# Autodesk Inventor assembly: fab_model_mk-2[1]
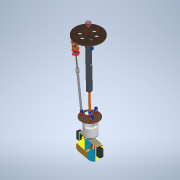
[picture p0: Inventor's stored thumbnail of the model, 180x180]
Saved by Autodesk Inventor 2021 (Build 250183000, 183)
## iProperties
Created: 2020-12-19
Part Number: fab_model_mk-2[1]
Document SubType Name: Assembly
Designer: Vikki
Author: Vikki
## Documents named in this file (31)
- E:\UG projects\CTF- projects\BOREWELL RESCUER\borewell rescuebot 2021\pll manipulator files\sps manipulator\fab_model_mk-2 scavenger bot.iam
- E:\UG projects\CTF- projects\BOREWELL RESCUER\borewell rescuebot 2021\pll manipulator files\sps manipulator\base.ipt
- E:\UG projects\CTF- projects\BOREWELL RESCUER\borewell rescuebot 2021\pll manipulator files\sps manipulator\craftsman-3-pc-universal-joint-set-1.snapshot.1\Craftsman Socket U-Joint.iam
- E:\UG projects\CTF- projects\BOREWELL RESCUER\borewell rescuebot 2021\pll manipulator files\sps manipulator\platform.ipt
- E:\UG projects\CTF- projects\BOREWELL RESCUER\borewell rescuebot 2021\pll manipulator files\sps manipulator\leadscrew.ipt
- E:\UG projects\CTF- projects\BOREWELL RESCUER\borewell rescuebot 2021\pll manipulator files\sps manipulator\coupler.ipt
- E:\UG projects\CTF- projects\BOREWELL RESCUER\borewell rescuebot 2021\pll manipulator files\sps manipulator\telescopic boom1.ipt
- E:\UG projects\CTF- projects\BOREWELL RESCUER\borewell rescuebot 2021\pll manipulator files\sps manipulator\boom 3.ipt
- E:\UG projects\CTF- projects\BOREWELL RESCUER\borewell rescuebot 2021\pll manipulator files\sps manipulator\ball-pin.ipt
- E:\UG projects\CTF- projects\BOREWELL RESCUER\borewell rescuebot 2021\2020 bot\borewell max sixe.ipt
- E:\UG projects\CTF- projects\BOREWELL RESCUER\borewell rescuebot 2021\2020 bot\min size bore well.ipt
- E:\UG projects\CTF- projects\BOREWELL RESCUER\borewell rescuebot 2021\pll manipulator files\sps manipulator\MicroGearmotor v3.ipt
- E:\UG projects\CTF- projects\BOREWELL RESCUER\borewell rescuebot 2021\pll manipulator files\sps manipulator\plunger.ipt
- E:\UG projects\CTF- projects\BOREWELL RESCUER\borewell rescuebot 2021\pll manipulator files\sps manipulator\piston.ipt
- E:\UG projects\CTF- projects\BOREWELL RESCUER\borewell rescuebot 2021\pll manipulator files\sps manipulator\motor bracket n 20.ipt
- E:\UG projects\CTF- projects\BOREWELL RESCUER\borewell rescuebot 2021\pll manipulator files\sps manipulator\female joint for uv.ipt
- E:\UG projects\CTF- projects\BOREWELL RESCUER\borewell rescuebot 2021\pll manipulator files\sps manipulator\platform uv femal joint.ipt
- E:\UG projects\CTF- projects\BOREWELL RESCUER\borewell rescuebot 2021\pll manipulator files\sps manipulator\boom to female.ipt
- E:\UG projects\CTF- projects\BOREWELL RESCUER\borewell rescuebot 2021\pll manipulator files\sps manipulator\fab_model_mk-2[1]\Design Accelerator\Bearing1.iam
- E:\UG projects\CTF- projects\BOREWELL RESCUER\borewell rescuebot 2021\pll manipulator files\sps manipulator\z axis-motor coupling.ipt
- E:\UG projects\CTF- projects\BOREWELL RESCUER\borewell rescuebot 2021\pll manipulator files\sps manipulator\jack-pin.ipt
- E:\UG projects\CTF- projects\BOREWELL RESCUER\borewell rescuebot 2021\pll manipulator files\sps manipulator\kiso.ipt
- E:\UG projects\CTF- projects\BOREWELL RESCUER\borewell rescuebot 2021\pll manipulator files\sps manipulator\new-motor-base.ipt
- E:\UG projects\CTF- projects\BOREWELL RESCUER\borewell rescuebot 2021\pll manipulator files\sps manipulator\end eff servo-conector.ipt
- E:\UG projects\CTF- projects\BOREWELL RESCUER\borewell rescuebot 2021\pll manipulator files\sps manipulator\clamshell half.ipt
- E:\UG projects\CTF- projects\BOREWELL RESCUER\borewell rescuebot 2021\pll manipulator files\sps manipulator\clamshell half-2.ipt
- E:\UG projects\CTF- projects\BOREWELL RESCUER\borewell rescuebot 2021\pll manipulator files\sps manipulator\clamshell cross link.ipt
- E:\UG projects\CTF- projects\BOREWELL RESCUER\borewell rescuebot 2021\pll manipulator files\sps manipulator\clamsheel sheet surface.ipt
- E:\UG projects\CTF- projects\BOREWELL RESCUER\borewell rescuebot 2021\pll manipulator files\sps manipulator\fab_model_mk-2[1]\Design Accelerator\Bearing3.iam
- E:\UG projects\CTF- projects\BOREWELL RESCUER\borewell rescuebot 2021\pll manipulator files\sps manipulator\n20 motor 3dp support.ipt
- E:\UG projects\CTF- projects\BOREWELL RESCUER\borewell rescuebot 2021\pll manipulator files\sps manipulator\z axis motor cover.ipt
## Components (45 placed, 29 different names)
1. base:1 — Mate:1, Mate:2, Mate:3, Mate:4, Mate:5, Mate:6, Angle:1, Mate:18, Mate:19, Mate:61, Flush:6, M1 C, M2 C, Mate:150, Mate:151
2. Craftsman Socket U-Joint:1 [sub-assembly] — Mate:1, Mate:2, Angle:2, Mate:90
3. Craftsman Socket U-Joint:2 [sub-assembly] — Mate:5, Mate:6, Angle:3, Mate:92
4. Craftsman Socket U-Joint:3 [sub-assembly] — Mate:3, Mate:4, Angle:1, Angle:2, Angle:3, Mate:23, Mate:91, Mate:93, Angle:7, Mate:108, Mate:109
5. platform:1 — Mate:7, Mate:9, Mate:10, Mate:16, Mate:17, M1 C, M2 C, Angle:6, Mate:134, Mate:135, Mate:136, Mate:199, Mate:200, Mate:201, Mate:204, Mate:205
6. Craftsman Socket U-Joint:4 [sub-assembly] — Mate:7, Mate:90, Mate:135
7. Craftsman Socket U-Joint:5 [sub-assembly] — Mate:9, Mate:91, Mate:111, Mate:112, Mate:136
8. Craftsman Socket U-Joint:6 [sub-assembly] — Mate:10, Mate:23, Mate:92, Mate:134
9. Craftsman Socket U-Joint:7 [sub-assembly] — Mate:16, Mate:17, Mate:26, Flush:1, Mate:60, Angle:6, Mate:100, Mate:101
10. Craftsman Socket U-Joint:8 [sub-assembly] — Mate:18, Mate:19, Angle:5, Mate:26, Flush:1, Mate:48, Mate:59, Mate:114, Mate:115
11. leadscrew:1 — Mate:97, Mate:167, Mate:187, Mate:188
12. telescopic boom1:1 — Mate:48, Mate:59, Angle:12
13. boom 3:1 — Mate:100, Mate:101, Angle:12
14. ball-pin:1 — Mate:60
15. borewell max sixe:1 — Mate:61, Mate:62, Flush:5
16. min size bore well:1 — Mate:62, Flush:5, Flush:6
17. MicroGearmotor v3:1 — Mate:93, Angle:7, Angle:9, Mate:120, Mate:167
18. plunger:1 — Mate:97, Angle:11, Mate:113, Mate:137
19. piston:1 — Angle:10, Angle:11, Mate:117
20. motor bracket n 20:1 — Angle:9, Mate:110, Angle:10, Mate:117, Mate:120, Flush:26, Mate:203
21. female joint for uv:1 — Mate:108, Mate:109, Mate:110
22. platform uv femal joint:1 — Mate:111, Mate:112, Mate:113, Mate:137
23. boom to female:1 — Mate:114, Mate:115
24. coupler:2 — Mate:188, Mate:189
25. Bearing:6 [sub-assembly] — Mate:187, Flush:26, Mate:189
26. z axis-motor coupling:1 — Mate:152, Mate:153, Mate:190, Mate:204, Mate:205
27. jack-pin:1 — Mate:150, Mate:151, Mate:191, Flush:27
28. kiso:1 — Mate:157, Mate:162, Mate:163, Mate:168, Mate:169, Mate:170
29. new-motor-base:1 — Mate:152, Mate:153, Mate:157, Mate:168, Mate:169, Mate:171, Mate:172, Mate:190, Angle:14
30. kiso:2 — Mate:160, Mate:161, Mate:170, Mate:171, Mate:172
31. end eff servo-conector:1 — Mate:160, Mate:161, Mate:173, Mate:174
32. end eff servo-conector:2 — Mate:162, Mate:163, Mate:165, Mate:166
33. clamshell half:1 — Flush:14, Mate:164, Mate:165, Mate:166, Flush:17, Mate:177, Mate:179, Mate:186, Flush:20, Flush:21
34. clamshell half-2:1 — Flush:14, Mate:164, Flush:16, Mate:180, Mate:181, Mate:182, Mate:183, Flush:18
35. clamshell half:2 — Mate:173, Mate:174, Mate:175, Flush:15, Flush:16, Flush:22, Flush:23, Flush:24, Flush:25, Angle:14, Mate:192
36. clamshell half-2:2 — Mate:175, Flush:15, Flush:17, Mate:184, Mate:185, Mate:192
37. clamshell cross link:1 — Mate:177, Mate:184
38. clamshell cross link:2 — Mate:179, Mate:185
39. clamshell cross link:3 — Mate:180, Mate:181
40. clamshell cross link:4 — Mate:182, Mate:183
41. clamsheel sheet surface:1 — Flush:18, Flush:22, Flush:23, Flush:24, Flush:25
42. clamsheel sheet surface:2 — Mate:186, Flush:20, Flush:21
43. Bearing:7 [sub-assembly] — Mate:191, Flush:27
44. n20 motor 3dp support:1 — Mate:203
45. z axis motor cover:1 — Mate:199, Mate:200, Mate:201
## Relationships (114: Mate 84, Flush 19, Angle 11)
- Mate:1: base:1 ↔ Craftsman Socket U-Joint:1
- Mate:2: base:1 ↔ Craftsman Socket U-Joint:1
- Mate:3: base:1 ↔ Craftsman Socket U-Joint:3
- Mate:4: base:1 ↔ Craftsman Socket U-Joint:3
- Mate:5: base:1 ↔ Craftsman Socket U-Joint:2
- Mate:6: base:1 ↔ Craftsman Socket U-Joint:2
- Mate:7: platform:1 ↔ Craftsman Socket U-Joint:4
- Mate:9: platform:1 ↔ Craftsman Socket U-Joint:5
- Mate:10: platform:1 ↔ Craftsman Socket U-Joint:6
- Angle:1 (30 deg): base:1 ↔ Craftsman Socket U-Joint:3
- Angle:2 (60 deg): Craftsman Socket U-Joint:1 ↔ Craftsman Socket U-Joint:3
- Angle:3 (120 deg): Craftsman Socket U-Joint:2 ↔ Craftsman Socket U-Joint:3
- Mate:16: platform:1 ↔ Craftsman Socket U-Joint:7
- Mate:17: platform:1 ↔ Craftsman Socket U-Joint:7
- Mate:18: base:1 ↔ Craftsman Socket U-Joint:8
- Mate:19: base:1 ↔ Craftsman Socket U-Joint:8
- Angle:5 (0 deg): Craftsman Socket U-Joint:8
- Mate:23: Craftsman Socket U-Joint:3 ↔ Craftsman Socket U-Joint:6
- Mate:26: Craftsman Socket U-Joint:7 ↔ Craftsman Socket U-Joint:8
- Flush:1: Craftsman Socket U-Joint:7 ↔ Craftsman Socket U-Joint:8
- Mate:48: Craftsman Socket U-Joint:8 ↔ telescopic boom1:1
- Mate:59 (-5 mm): Craftsman Socket U-Joint:8 ↔ telescopic boom1:1
- Mate:60: Craftsman Socket U-Joint:7 ↔ ball-pin:1
- [Flush]: borewell max sixe:1 ↔ min size bore well:1
- [Flush]: borewell max sixe:1 ↔ min size bore well:1
- Mate:61: base:1 ↔ borewell max sixe:1
- Mate:62: borewell max sixe:1 ↔ min size bore well:1
- Flush:5: borewell max sixe:1 ↔ min size bore well:1
- Flush:6 (-400 mm): base:1 ↔ min size bore well:1
- M1 C [Flush] (400 mm): base:1 ↔ platform:1
- M2 C [Mate]: base:1 ↔ platform:1
- Mate:90: Craftsman Socket U-Joint:1 ↔ Craftsman Socket U-Joint:4
- Mate:91: Craftsman Socket U-Joint:3 ↔ Craftsman Socket U-Joint:5
- Mate:92: Craftsman Socket U-Joint:2 ↔ Craftsman Socket U-Joint:6
- Angle:6 (30 deg): platform:1 ↔ Craftsman Socket U-Joint:7
- Mate:93: Craftsman Socket U-Joint:3 ↔ MicroGearmotor v3:1
- Angle:7 (0 deg): Craftsman Socket U-Joint:3 ↔ MicroGearmotor v3:1
- Mate:97: leadscrew:1 ↔ plunger:1
- Mate:100: Craftsman Socket U-Joint:7 ↔ boom 3:1
- Mate:101: Craftsman Socket U-Joint:7 ↔ boom 3:1
- Angle:9 (0 deg): MicroGearmotor v3:1 ↔ motor bracket n 20:1
- Mate:108: Craftsman Socket U-Joint:3 ↔ female joint for uv:1
- Mate:109: Craftsman Socket U-Joint:3 ↔ female joint for uv:1
- Mate:110: motor bracket n 20:1 ↔ female joint for uv:1
- Angle:10 (0 deg): piston:1 ↔ motor bracket n 20:1
- Angle:11 (0 deg): plunger:1 ↔ piston:1
- Mate:111: Craftsman Socket U-Joint:5 ↔ platform uv femal joint:1
- Mate:112: Craftsman Socket U-Joint:5 ↔ platform uv femal joint:1
- Mate:113: plunger:1 ↔ platform uv femal joint:1
- Angle:12 (0 deg): telescopic boom1:1 ↔ boom 3:1
- Mate:114: Craftsman Socket U-Joint:8 ↔ boom to female:1
- Mate:115: Craftsman Socket U-Joint:8 ↔ boom to female:1
- Mate:117: piston:1 ↔ motor bracket n 20:1
- Mate:120: MicroGearmotor v3:1 ↔ motor bracket n 20:1
- Mate:134: platform:1 ↔ Craftsman Socket U-Joint:6
- Mate:135: platform:1 ↔ Craftsman Socket U-Joint:4
- Mate:136: platform:1 ↔ Craftsman Socket U-Joint:5
- Mate:137: plunger:1 ↔ platform uv femal joint:1
- Mate:150: base:1 ↔ jack-pin:1
- Mate:151: base:1 ↔ jack-pin:1
- Mate:152: z axis-motor coupling:1 ↔ new-motor-base:1
- Mate:153: z axis-motor coupling:1 ↔ new-motor-base:1
- Mate:157: kiso:1 ↔ new-motor-base:1
- Mate:160: kiso:2 ↔ end eff servo-conector:1
- Mate:161 (0.5 mm): kiso:2 ↔ end eff servo-conector:1
- Mate:162: kiso:1 ↔ end eff servo-conector:2
- Mate:163 (0.5 mm): kiso:1 ↔ end eff servo-conector:2
- Flush:14: clamshell half:1 ↔ clamshell half-2:1
- Mate:164: clamshell half:1 ↔ clamshell half-2:1
- Mate:165: end eff servo-conector:2 ↔ clamshell half:1
- Mate:166: end eff servo-conector:2 ↔ clamshell half:1
- Mate:167: leadscrew:1 ↔ MicroGearmotor v3:1
- Mate:168: kiso:1 ↔ new-motor-base:1
- Mate:169: kiso:1 ↔ new-motor-base:1
- Mate:170: kiso:1 ↔ kiso:2
- Mate:171: new-motor-base:1 ↔ kiso:2
- Mate:172: new-motor-base:1 ↔ kiso:2
- Mate:173: end eff servo-conector:1 ↔ clamshell half:2
- Mate:174: end eff servo-conector:1 ↔ clamshell half:2
- Mate:175: clamshell half:2 ↔ clamshell half-2:2
- Flush:15: clamshell half:2 ↔ clamshell half-2:2
- Flush:16: clamshell half-2:1 ↔ clamshell half:2
- Flush:17: clamshell half:1 ↔ clamshell half-2:2
- Mate:177: clamshell half:1 ↔ clamshell cross link:1
- Mate:179: clamshell half:1 ↔ clamshell cross link:2
- Mate:180: clamshell half-2:1 ↔ clamshell cross link:3
- Mate:181: clamshell half-2:1 ↔ clamshell cross link:3
- Mate:182: clamshell half-2:1 ↔ clamshell cross link:4
- Mate:183: clamshell half-2:1 ↔ clamshell cross link:4
- Mate:184: clamshell half-2:2 ↔ clamshell cross link:1
- Mate:185: clamshell half-2:2 ↔ clamshell cross link:2
- Flush:18: clamshell half-2:1 ↔ clamsheel sheet surface:1
- Mate:186: clamshell half:1 ↔ clamsheel sheet surface:2
- Flush:20: clamshell half:1 ↔ clamsheel sheet surface:2
- Flush:21: clamshell half:1 ↔ clamsheel sheet surface:2
- Flush:22: clamshell half:2 ↔ clamsheel sheet surface:1
- Flush:23: clamshell half:2 ↔ clamsheel sheet surface:1
- Flush:24: clamshell half:2 ↔ clamsheel sheet surface:1
- Flush:25: clamshell half:2 ↔ clamsheel sheet surface:1
- Mate:187: leadscrew:1 ↔ Bearing:6
- Flush:26: motor bracket n 20:1 ↔ Bearing:6
- Mate:188: leadscrew:1 ↔ coupler:2
- Mate:189: coupler:2 ↔ Bearing:6
- Mate:190: z axis-motor coupling:1 ↔ new-motor-base:1
- Mate:191: jack-pin:1 ↔ Bearing:7
- Flush:27: jack-pin:1 ↔ Bearing:7
- Angle:14 (0 deg): new-motor-base:1 ↔ clamshell half:2
- Mate:192: clamshell half:2 ↔ clamshell half-2:2
- Mate:199: platform:1 ↔ z axis motor cover:1
- Mate:200: platform:1 ↔ z axis motor cover:1
- Mate:201: platform:1 ↔ z axis motor cover:1
- Mate:203: motor bracket n 20:1 ↔ n20 motor 3dp support:1
- Mate:204: platform:1 ↔ z axis-motor coupling:1
- Mate:205 (3 mm): platform:1 ↔ z axis-motor coupling:1
